# Autodesk Inventor assembly: CanSat
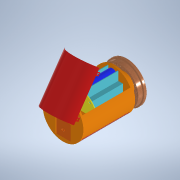
[picture p0: Inventor's stored thumbnail of the model, 180x180]
Saved by Autodesk Inventor 2020 (Build 240168000, 168)
## iProperties
Created: 2021-10-14
Part Number: CanSat
Document SubType Name: Assembly
Designer: Komputer
Author: Komputer
## Documents named in this file (16)
- C:\Users\Komputer\Documents\Inventor\Satcan\CanSat.iam
- C:\Users\Komputer\Documents\Inventor\Satcan\Część5.ipt
- C:\Users\Komputer\Documents\Inventor\Satcan\Mocowanie spadochronu.ipt
- C:\Users\Komputer\Documents\Inventor\Content Center Files\R2020\pl-PL\CSN 024665 SKF (A)\CSN 024665 SKF (A) - SKF 3200 A.ipt
- C:\Users\Komputer\Documents\Inventor\Satcan\Korpus.ipt
- C:\Users\Komputer\Documents\Inventor\Satcan\Silnik krokowy.ipt
- C:\Users\Komputer\Documents\Inventor\Satcan\Zestaw startowy Cansat.ipt
- C:\Users\Komputer\Documents\Inventor\Satcan\Czujnik AltIMU-10.ipt
- C:\Users\Komputer\Documents\Inventor\Satcan\Czujnik BMP280.ipt
- C:\Users\Komputer\Documents\Inventor\Satcan\Czujnik GPS ZOE-M8Q.ipt
- C:\Users\Komputer\Documents\Inventor\Satcan\Kamera.ipt
- C:\Users\Komputer\Documents\Inventor\Satcan\Bateria.ipt
- C:\Users\Komputer\Documents\Inventor\Satcan\Magazynek na baterie.ipt
- C:\Users\Komputer\Documents\Inventor\Satcan\Termopara.ipt
- C:\Users\Komputer\Documents\Inventor\Satcan\Obudowa, większa.ipt
- C:\Users\Komputer\Documents\Inventor\Satcan\Obudowa, mniejsza.ipt
## Components (17 placed, 15 different names)
1. Korpus:1 — Zestawiające:1, Styczny:1, Równoległe:1, Zestawiające:2, Zestawiające:3, Zestawiające:7, Zestawiające:8, Zestawiające:9, Zestawiające:10, Zestawiające:11, Zestawiające:12, Zestawiające:14, Kątowe:1, Zestawiające:15, Zestawiające:16, Zestawiające:17, Równoległe:2, Zestawiające:18, Zestawiające:19, Zestawiające:23, Styczny:8, Zestawiające:24, Zestawiające:26, Zestawiające:27, Zestawiające:28, Zestawiające:29
2. CSN 024665 SKF SKF 3200 A:1 — Zestawiające:1, Styczny:1, Zestawiające:6
3. Silnik krokowy:1 — Równoległe:1, Zestawiające:2, Zestawiające:3, Zestawiające:4, Zestawiające:5
4. Część5:1 — Zestawiające:4, Zestawiające:5
5. Mocowanie spadochronu:1 — Zestawiające:6, Zestawiające:7
6. Czujnik AltIMU-10:1 — Zestawiające:8, Zestawiające:9
7. Czujnik GPS ZOE-M8Q:1 — Zestawiające:10
8. Czujnik BMP280:1 — Zestawiające:11, Zestawiające:12
9. Zestaw startowy Cansat:1 — Zestawiające:14, Kątowe:1, Zestawiające:15
10. Kamera:1 — Zestawiające:16, Zestawiające:17, Równoległe:2
11. Magazynek na baterie:1 — Zestawiające:18, Zestawiające:19, Zestawiające:20, Styczny:2, Styczny:3, Zestawiające:21, Styczny:4, Styczny:5, Zestawiające:22, Styczny:6, Styczny:7, Zestawiające:23
12. Bateria:1 — Zestawiające:20, Styczny:2, Styczny:3
13. Bateria:2 — Zestawiające:21, Styczny:4, Styczny:5
14. Bateria:3 — Zestawiające:22, Styczny:6, Styczny:7
15. Termopara:1 — Styczny:8, Zestawiające:24
16. Obudowa, większa:1 — Zestawiające:26, Zestawiające:27
17. Obudowa, mniejsza:1 — Zestawiające:28, Zestawiające:29
## Relationships (38: Mate 27, Tangent 8, Flush 2, Angle 1)
- Zestawiające:1 [Mate] (0.5 mm): Korpus:1 ↔ CSN 024665 SKF SKF 3200 A:1
- Styczny:1 [Tangent]: Korpus:1 ↔ CSN 024665 SKF SKF 3200 A:1
- Równoległe:1 [Flush] (1 mm): Korpus:1 ↔ Silnik krokowy:1
- Zestawiające:2 [Mate]: Korpus:1 ↔ Silnik krokowy:1
- Zestawiające:3 [Mate]: Korpus:1 ↔ Silnik krokowy:1
- Zestawiające:4 [Mate]: Silnik krokowy:1 ↔ Część5:1
- Zestawiające:5 [Mate]: Silnik krokowy:1 ↔ Część5:1
- Zestawiające:6 [Mate]: CSN 024665 SKF SKF 3200 A:1 ↔ Mocowanie spadochronu:1
- Zestawiające:7 [Mate] (0.5 mm): Korpus:1 ↔ Mocowanie spadochronu:1
- Zestawiające:8 [Mate]: Korpus:1 ↔ Czujnik AltIMU-10:1
- Zestawiające:9 [Mate]: Korpus:1 ↔ Czujnik AltIMU-10:1
- Zestawiające:10 [Mate]: Korpus:1 ↔ Czujnik GPS ZOE-M8Q:1
- Zestawiające:11 [Mate]: Korpus:1 ↔ Czujnik BMP280:1
- Zestawiające:12 [Mate]: Korpus:1 ↔ Czujnik BMP280:1
- Zestawiające:14 [Mate]: Korpus:1 ↔ Zestaw startowy Cansat:1
- Kątowe:1 [Angle] (0 deg): Korpus:1 ↔ Zestaw startowy Cansat:1
- Zestawiające:15 [Mate] (1 mm): Korpus:1 ↔ Zestaw startowy Cansat:1
- Zestawiające:16 [Mate]: Korpus:1 ↔ Kamera:1
- Zestawiające:17 [Mate]: Korpus:1 ↔ Kamera:1
- Równoległe:2 [Flush]: Korpus:1 ↔ Kamera:1
- Zestawiające:18 [Mate] (-1 mm): Korpus:1 ↔ Magazynek na baterie:1
- Zestawiające:19 [Mate]: Korpus:1 ↔ Magazynek na baterie:1
- Zestawiające:20 [Mate]: Magazynek na baterie:1 ↔ Bateria:1
- Styczny:2 [Tangent] (0.5 mm): Magazynek na baterie:1 ↔ Bateria:1
- Styczny:3 [Tangent]: Magazynek na baterie:1 ↔ Bateria:1
- Zestawiające:21 [Mate]: Magazynek na baterie:1 ↔ Bateria:2
- Styczny:4 [Tangent]: Magazynek na baterie:1 ↔ Bateria:2
- Styczny:5 [Tangent] (0.5 mm): Magazynek na baterie:1 ↔ Bateria:2
- Zestawiające:22 [Mate]: Magazynek na baterie:1 ↔ Bateria:3
- Styczny:6 [Tangent] (0.5 mm): Magazynek na baterie:1 ↔ Bateria:3
- Styczny:7 [Tangent]: Magazynek na baterie:1 ↔ Bateria:3
- Zestawiające:23 [Mate] (19.5 mm): Korpus:1 ↔ Magazynek na baterie:1
- Styczny:8 [Tangent]: Korpus:1 ↔ Termopara:1
- Zestawiające:24 [Mate]: Korpus:1 ↔ Termopara:1
- Zestawiające:26 [Mate]: Korpus:1 ↔ Obudowa, większa:1
- Zestawiające:27 [Mate]: Korpus:1 ↔ Obudowa, większa:1
- Zestawiające:28 [Mate]: Korpus:1 ↔ Obudowa, mniejsza:1
- Zestawiające:29 [Mate]: Korpus:1 ↔ Obudowa, mniejsza:1
